# Autodesk Inventor assembly: Assembly1
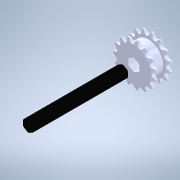
[picture p0: Inventor's stored thumbnail of the model, 180x180]
Saved by Autodesk Inventor 2020 (Build 240168000, 168)
## iProperties
Created: 2021-01-23
Part Number: Assembly1
Document SubType Name: Assembly
Designer: magda
Author: magda
## Documents named in this file (3)
- C:\Users\magda\OneDrive\Documents\Inventor\T3\Glock\Assembly1.iam
- C:\Users\magda\Downloads\5.5 thundershaft.ipt
- C:\Users\magda\Downloads\15T Double Sprocket.ipt
## Components (2 placed, 2 different names)
1. 5.5 thundershaft:1 — Mate:1, Mate:2
2. 15T Double Sprocket:1 — Mate:1, Mate:2
## Relationships (2: Mate 2)
- Mate:1 (0.0127 mm): 5.5 thundershaft:1 ↔ 15T Double Sprocket:1
- Mate:2 (0.0127 mm): 5.5 thundershaft:1 ↔ 15T Double Sprocket:1
